# Autodesk Inventor assembly: WheelModule
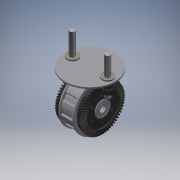
[picture p0: Inventor's stored thumbnail of the model, 180x180]
Saved by Autodesk Inventor 2019.3 (Build 233278000, 278)
## iProperties
Created: 2019-04-08
Part Number: WheelModule
Document SubType Name: Assembly
Designer: Connor
Author: Connor
## Documents named in this file (8)
- C:\Users\Connor\Documents\GrabCAD\NuSwerve\WheelModule.iam
- C:\Users\Connor\Documents\GrabCAD\NuSwerve\Imported Components\Wheels and Hubs\VEX Traction Wheels\TractionWheel 4x1\TractionWheel 4x1.iam
- C:\Users\Connor\Documents\GrabCAD\NuSwerve\15t_bevel.ipt
- C:\Users\Connor\Documents\GrabCAD\NuSwerve\60t_bevel.ipt
- C:\Users\Connor\Documents\GrabCAD\NuSwerve\Imported Components\Bearings\0_500_ID_x_1_125_OD_x_0_313_WD_Flanged_Bearing_217-2731.ipt
- C:\Users\Connor\Documents\GrabCAD\NuSwerve\Imported Components\Bearings\10_25mm_3_8_ThunderHex_ID_x_0_875_OD_x_0_280_WD_Flanged_Bearing_217-5829.ipt
- C:\Users\Connor\Documents\GrabCAD\NuSwerve\drive_shaft.ipt
- C:\Users\Connor\Documents\GrabCAD\NuSwerve\main_plate.ipt
## Components (12 placed, 7 different names)
1. TractionWheel 4x1:1 [sub-assembly] — Mate:5, Mate:6, Mate:8, Mate:9, Mate:13, Mate:14
2. 15t_bevel:1 — Tangent:1, Mate:10, Flush:1, Mate:19, Mate:21, Mate:25
3. 60t_bevel:1 — Mate:5, Mate:6, Tangent:1, Mate:10, Flush:1, Mate:13, Mate:15, Mate:16
4. 15t_bevel:2 — Mate:12, Flush:2, Tangent:2, Mate:20, Mate:22, Mate:26
5. 60t_bevel:2 — Mate:8, Mate:9, Mate:12, Flush:2, Tangent:2, Mate:14, Mate:17, Mate:18
6. 0_500_ID_x_1_125_OD_x_0_313_WD_Flanged_Bearing_217-2731:1 — Mate:17, Mate:18
7. 0_500_ID_x_1_125_OD_x_0_313_WD_Flanged_Bearing_217-2731:2 — Mate:15, Mate:16
8. 10_25mm_3_8_ThunderHex_ID_x_0_875_OD_x_0_280_WD_Flanged_Bearing_217-5829:1 — Mate:19, Mate:21, Mate:23, Mate:29
9. 10_25mm_3_8_ThunderHex_ID_x_0_875_OD_x_0_280_WD_Flanged_Bearing_217-5829:2 — Mate:20, Mate:22, Mate:24
10. drive_shaft:1 — Mate:23, Mate:25
11. drive_shaft:2 — Mate:24, Mate:26
12. main_plate:1 — Mate:27, Mate:28, Mate:29
## Relationships (27: Mate 23, Tangent 2, Flush 2)
- Mate:5: TractionWheel 4x1:1 ↔ 60t_bevel:1
- Mate:6: TractionWheel 4x1:1 ↔ 60t_bevel:1
- Mate:8: TractionWheel 4x1:1 ↔ 60t_bevel:2
- Mate:9: TractionWheel 4x1:1 ↔ 60t_bevel:2
- Tangent:1 (11 mm): 15t_bevel:1 ↔ 60t_bevel:1
- Mate:10: 15t_bevel:1 ↔ 60t_bevel:1
- Flush:1 (-56 mm): 15t_bevel:1 ↔ 60t_bevel:1
- Mate:12 (-56 mm): 15t_bevel:2 ↔ 60t_bevel:2
- Flush:2: 15t_bevel:2 ↔ 60t_bevel:2
- Tangent:2 (11 mm): 15t_bevel:2 ↔ 60t_bevel:2
- Mate:13: TractionWheel 4x1:1 ↔ 60t_bevel:1
- Mate:14: TractionWheel 4x1:1 ↔ 60t_bevel:2
- Mate:15: 60t_bevel:1 ↔ 0_500_ID_x_1_125_OD_x_0_313_WD_Flanged_Bearing_217-2731:2
- Mate:16: 60t_bevel:1 ↔ 0_500_ID_x_1_125_OD_x_0_313_WD_Flanged_Bearing_217-2731:2
- Mate:17: 60t_bevel:2 ↔ 0_500_ID_x_1_125_OD_x_0_313_WD_Flanged_Bearing_217-2731:1
- Mate:18: 60t_bevel:2 ↔ 0_500_ID_x_1_125_OD_x_0_313_WD_Flanged_Bearing_217-2731:1
- Mate:19: 15t_bevel:1 ↔ 10_25mm_3_8_ThunderHex_ID_x_0_875_OD_x_0_280_WD_Flanged_Bearing_217-5829:1
- Mate:20: 15t_bevel:2 ↔ 10_25mm_3_8_ThunderHex_ID_x_0_875_OD_x_0_280_WD_Flanged_Bearing_217-5829:2
- Mate:21: 15t_bevel:1 ↔ 10_25mm_3_8_ThunderHex_ID_x_0_875_OD_x_0_280_WD_Flanged_Bearing_217-5829:1
- Mate:22: 15t_bevel:2 ↔ 10_25mm_3_8_ThunderHex_ID_x_0_875_OD_x_0_280_WD_Flanged_Bearing_217-5829:2
- Mate:23: 10_25mm_3_8_ThunderHex_ID_x_0_875_OD_x_0_280_WD_Flanged_Bearing_217-5829:1 ↔ drive_shaft:1
- Mate:24: 10_25mm_3_8_ThunderHex_ID_x_0_875_OD_x_0_280_WD_Flanged_Bearing_217-5829:2 ↔ drive_shaft:2
- Mate:25: 15t_bevel:1 ↔ drive_shaft:1
- Mate:26: 15t_bevel:2 ↔ drive_shaft:2
- Mate:27: main_plate:1
- Mate:28: main_plate:1
- Mate:29: 10_25mm_3_8_ThunderHex_ID_x_0_875_OD_x_0_280_WD_Flanged_Bearing_217-5829:1 ↔ main_plate:1
